# Autodesk Inventor assembly: 217-2799.20121203NEW
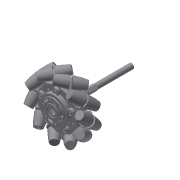
[picture p0: Inventor's stored thumbnail of the model, 180x180]
Saved by Autodesk Inventor 2015 (Build 190159000, 159)
## iProperties
Created: 2013-01-18
Part Number: 217-2799.20121203NEW
Document SubType Name: Assembly
Designer: Tanner
Author: Tanner
## Documents named in this file (12)
- T:\FILES\Inventor 2015 Projects\2013 Robot - Ultimate Ascent\Chassis - Wheel.iam
- T:\FILES\Inventor 2015 Projects\2013 Robot - Ultimate Ascent\Chassis - Wheel - 217-2799-001 Rev1.ipt
- T:\FILES\Inventor 2015 Projects\2013 Robot - Ultimate Ascent\Chassis - Wheel - 217-2799-002 Rev1.ipt
- T:\FILES\Inventor 2015 Projects\2013 Robot - Ultimate Ascent\Chassis - Wheel - 217-2586-003 Rev2.ipt
- T:\FILES\Inventor 2015 Projects\2013 Robot - Ultimate Ascent\Chassis - Wheel - 217-2586-004 Rev1.ipt
- T:\FILES\Inventor 2015 Projects\2013 Robot - Ultimate Ascent\Chassis - Wheel - 217-2586-007 Rev1.ipt
- T:\FILES\Inventor 2015 Projects\2013 Robot - Ultimate Ascent\Chassis - Wheel - 217-2586-008 Rev1.ipt
- T:\FILES\Inventor 2015 Projects\2013 Robot - Ultimate Ascent\Chassis - Wheel - NUT-832-NYLOCK.ipt
- T:\FILES\Inventor 2015 Projects\2013 Robot - Ultimate Ascent\Chassis - Wheel - SCREW-832-1250.ipt
- T:\FILES\Inventor 2015 Projects\2013 Robot - Ultimate Ascent\Chassis - Wheel - 217-2586-005 Rev2.ipt
- T:\FILES\Inventor 2015 Projects\2013 Robot - Ultimate Ascent\Chassis - Wheel - Versahub.ipt
- T:\FILES\Inventor 2015 Projects\2013 Robot - Ultimate Ascent\Chassis - Wheel - Shaft.ipt
## Components (101 placed, 11 different names)
1. Chassis - Wheel - 217-2799-001 Rev1:1 — Mate:3, Mate:4
2. Chassis - Wheel - 217-2799-001 Rev1:2 — Mate:1, Mate:2
3. Chassis - Wheel - 217-2799-002 Rev1:1
4. Chassis - Wheel - 217-2586-003 Rev2:1
5. Chassis - Wheel - 217-2586-003 Rev2:2
6. Chassis - Wheel - 217-2586-004 Rev1:1
7. Chassis - Wheel - 217-2586-004 Rev1:2
8. Chassis - Wheel - 217-2586-007 Rev1:1
9. Chassis - Wheel - 217-2586-008 Rev1:1
10. Chassis - Wheel - NUT-832-NYLOCK:1
11. Chassis - Wheel - SCREW-832-1250:1
12. Chassis - Wheel - 217-2586-007 Rev1:2
13. Chassis - Wheel - 217-2586-007 Rev1:3
14. Chassis - Wheel - 217-2586-007 Rev1:4
15. Chassis - Wheel - 217-2586-007 Rev1:5
16. Chassis - Wheel - 217-2586-007 Rev1:6
17. Chassis - Wheel - 217-2586-007 Rev1:7
18. Chassis - Wheel - 217-2586-007 Rev1:8
19. Chassis - Wheel - 217-2586-007 Rev1:9
20. Chassis - Wheel - 217-2586-007 Rev1:10
21. Chassis - Wheel - 217-2586-004 Rev1:3
22. Chassis - Wheel - 217-2586-004 Rev1:4
23. Chassis - Wheel - 217-2586-004 Rev1:5
24. Chassis - Wheel - 217-2586-004 Rev1:6
25. Chassis - Wheel - 217-2586-004 Rev1:7
26. Chassis - Wheel - 217-2586-004 Rev1:8
27. Chassis - Wheel - 217-2586-004 Rev1:9
28. Chassis - Wheel - 217-2586-004 Rev1:10
29. Chassis - Wheel - 217-2586-004 Rev1:11
30. Chassis - Wheel - 217-2586-004 Rev1:12
31. Chassis - Wheel - 217-2586-004 Rev1:13
32. Chassis - Wheel - 217-2586-004 Rev1:14
33. Chassis - Wheel - 217-2586-004 Rev1:15
34. Chassis - Wheel - 217-2586-004 Rev1:16
35. Chassis - Wheel - 217-2586-004 Rev1:17
36. Chassis - Wheel - 217-2586-004 Rev1:18
37. Chassis - Wheel - 217-2586-004 Rev1:19
38. Chassis - Wheel - 217-2586-004 Rev1:20
39. Chassis - Wheel - 217-2586-003 Rev2:3
40. Chassis - Wheel - 217-2586-003 Rev2:4
41. Chassis - Wheel - 217-2586-003 Rev2:5
42. Chassis - Wheel - 217-2586-003 Rev2:6
43. Chassis - Wheel - 217-2586-003 Rev2:7
44. Chassis - Wheel - 217-2586-003 Rev2:8
45. Chassis - Wheel - 217-2586-003 Rev2:9
46. Chassis - Wheel - 217-2586-003 Rev2:10
47. Chassis - Wheel - 217-2586-003 Rev2:11
48. Chassis - Wheel - 217-2586-003 Rev2:12
49. Chassis - Wheel - 217-2586-003 Rev2:13
50. Chassis - Wheel - 217-2586-003 Rev2:14
51. Chassis - Wheel - 217-2586-003 Rev2:15
52. Chassis - Wheel - 217-2586-003 Rev2:16
53. Chassis - Wheel - 217-2586-003 Rev2:17
54. Chassis - Wheel - 217-2586-003 Rev2:18
55. Chassis - Wheel - 217-2586-003 Rev2:19
56. Chassis - Wheel - 217-2586-003 Rev2:20
57. Chassis - Wheel - 217-2799-002 Rev1:2
58. Chassis - Wheel - 217-2799-002 Rev1:3
59. Chassis - Wheel - 217-2799-002 Rev1:4
60. Chassis - Wheel - 217-2799-002 Rev1:5
61. Chassis - Wheel - 217-2799-002 Rev1:6
62. Chassis - Wheel - 217-2799-002 Rev1:7
63. Chassis - Wheel - 217-2799-002 Rev1:8
64. Chassis - Wheel - 217-2799-002 Rev1:9
65. Chassis - Wheel - 217-2799-002 Rev1:10
66. Chassis - Wheel - 217-2586-008 Rev1:2
67. Chassis - Wheel - 217-2586-008 Rev1:3
68. Chassis - Wheel - 217-2586-008 Rev1:4
69. Chassis - Wheel - 217-2586-008 Rev1:5
70. Chassis - Wheel - 217-2586-008 Rev1:6
71. Chassis - Wheel - SCREW-832-1250:2
72. Chassis - Wheel - SCREW-832-1250:3
73. Chassis - Wheel - SCREW-832-1250:4
74. Chassis - Wheel - SCREW-832-1250:5
75. Chassis - Wheel - NUT-832-NYLOCK:2
76. Chassis - Wheel - NUT-832-NYLOCK:3
77. Chassis - Wheel - NUT-832-NYLOCK:4
78. Chassis - Wheel - NUT-832-NYLOCK:5
79. Chassis - Wheel - 217-2586-005 Rev2:1
80. Chassis - Wheel - 217-2586-005 Rev2:2
81. Chassis - Wheel - 217-2586-005 Rev2:3
82. Chassis - Wheel - 217-2586-005 Rev2:4
83. Chassis - Wheel - 217-2586-005 Rev2:5
84. Chassis - Wheel - 217-2586-005 Rev2:6
85. Chassis - Wheel - 217-2586-005 Rev2:7
86. Chassis - Wheel - 217-2586-005 Rev2:8
87. Chassis - Wheel - 217-2586-005 Rev2:9
88. Chassis - Wheel - 217-2586-005 Rev2:10
89. Chassis - Wheel - 217-2586-005 Rev2:11
90. Chassis - Wheel - 217-2586-005 Rev2:12
91. Chassis - Wheel - 217-2586-005 Rev2:13
92. Chassis - Wheel - 217-2586-005 Rev2:14
93. Chassis - Wheel - 217-2586-005 Rev2:15
94. Chassis - Wheel - 217-2586-005 Rev2:16
95. Chassis - Wheel - 217-2586-005 Rev2:17
96. Chassis - Wheel - 217-2586-005 Rev2:18
97. Chassis - Wheel - 217-2586-005 Rev2:19
98. Chassis - Wheel - 217-2586-005 Rev2:20
99. Chassis - Wheel - Versahub:1 — Mate:3, Mate:4, Angle:1
100. Chassis - Wheel - Versahub:2 — Mate:1, Mate:2, Mate:5, Mate:6, Angle:1
101. Chassis - Wheel - Shaft:1 — Mate:5, Mate:6
## Relationships (7: Mate 6, Angle 1)
- Mate:1: Chassis - Wheel - 217-2799-001 Rev1:2 ↔ Chassis - Wheel - Versahub:2
- Mate:2: Chassis - Wheel - 217-2799-001 Rev1:2 ↔ Chassis - Wheel - Versahub:2
- Mate:3: Chassis - Wheel - 217-2799-001 Rev1:1 ↔ Chassis - Wheel - Versahub:1
- Mate:4: Chassis - Wheel - 217-2799-001 Rev1:1 ↔ Chassis - Wheel - Versahub:1
- Mate:5: Chassis - Wheel - Versahub:2 ↔ Chassis - Wheel - Shaft:1
- Mate:6: Chassis - Wheel - Versahub:2 ↔ Chassis - Wheel - Shaft:1
- Angle:1 (0 deg): Chassis - Wheel - Versahub:1 ↔ Chassis - Wheel - Versahub:2
